# Autodesk Inventor assembly: yaw_unit_mir
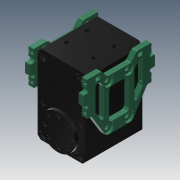
[picture p0: Inventor's stored thumbnail of the model, 180x180]
Saved by Autodesk Inventor 2018 (Build 220112000, 112)
## iProperties
Created: 2018-08-06
Part Number: yaw_unit_mir
Material: 一般
Document SubType Name: Assembly
Designer: student
Author: student
## Documents named in this file (4)
- C:\Users\y6tada\Dropbox\曹研究室\多田\Intel NUC Hexapod\Inventor\Thorax\yaw_unit\yaw_unit_mir.iam
- C:\Users\y6tada\Dropbox\曹研究室\多田\Intel NUC Hexapod\Inventor\X430\XL-430_mir.iam
- C:\Users\y6tada\Dropbox\曹研究室\多田\Intel NUC Hexapod\Inventor\Thorax\yaw_unit\yaw_servo_side_mir2.ipt
- C:\Users\y6tada\Dropbox\曹研究室\多田\Intel NUC Hexapod\Inventor\Thorax\yaw_unit\yaw_servo_side_mir1_mir.ipt
## Components (3 placed, 3 different names)
1. XL-430_mir:1 [sub-assembly] — フラッシュ:2, メイト:4, フラッシュ:1, メイト:3, メイト:2, メイト:1
2. yaw_servo_side_mir2:1 — メイト:3, メイト:2, メイト:1
3. yaw_servo_side_mir1_mir:1
## Relationships (6: Mate 4, Flush 2)
- フラッシュ:2 [Mate]: XL-430_mir:1
- メイト:4 [Flush]: XL-430_mir:1
- フラッシュ:1 [Flush]: XL-430_mir:1
- メイト:3 [Mate]: XL-430_mir:1 ↔ yaw_servo_side_mir2:1
- メイト:2 [Mate]: XL-430_mir:1 ↔ yaw_servo_side_mir2:1
- メイト:1 [Mate]: XL-430_mir:1 ↔ yaw_servo_side_mir2:1
